# Autodesk Inventor assembly: KND-3600 Branch 6 01
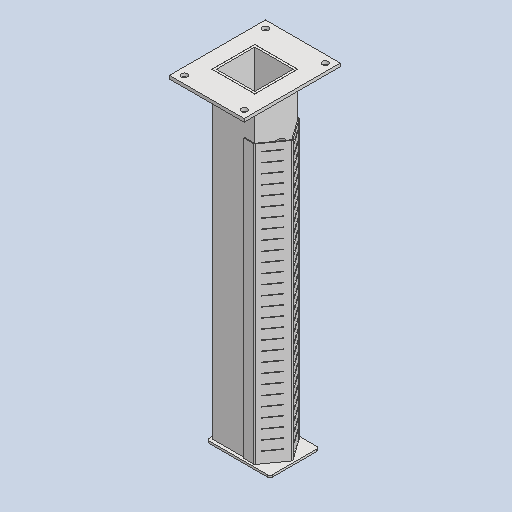
[picture p0: Inventor's stored thumbnail of the model, 512x512]
Saved by Autodesk Inventor 2026.2 (Build 302298000, 298)
## iProperties
Created: 2026-10-05
Part Number: KND-3600 Branch 6 01
Document SubType Name: Assembly
Designer: admin
Stock Number: Луч 6
Author: admin
## Documents named in this file (5)
- C:\Users\admin\Documents\Inventor\KND-DistribSystem\DRS_D1200\KND-3600 Branch 6 01.iam
- C:\Users\admin\Documents\Inventor\KND-DistribSystem\DRS_D1200\KND-1668 DrSysB way tube 6 01.ipt
- C:\Users\admin\Documents\Inventor\KND-DistribSystem\DRS_D1200\KND-1425 DrSysB Way FLANGE 01.ipt
- C:\Users\admin\Documents\Inventor\KND-DistribSystem\DRS_D1200\KND-5338 DrSysB roof 6 01.ipt
- C:\Users\admin\Documents\Inventor\KND-DistribSystem\DRS_D1200\KND-1666 FDS 1000 CUP 1 01.ipt
## Components (4 placed, 4 different names)
1. KND-1668 DrSysB way tube 6 01:1 — Flush:1, Mate:1, Mate:2, Flush:2, Mate:3, Mate:4, Mate:5, Flush:3, Flush:4
2. KND-1425 DrSysB Way FLANGE 01:1 — Flush:1, Mate:1, Mate:2
3. KND-5338 DrSysB roof 6 01:1 — Flush:2, Mate:3, Mate:4
4. KND-1666 FDS 1000 CUP 1 01:1 — Mate:5, Flush:3, Flush:4
## Relationships (9: Mate 5, Flush 4)
- Flush:1: KND-1668 DrSysB way tube 6 01:1 ↔ KND-1425 DrSysB Way FLANGE 01:1
- Mate:1 (0.1 mm): KND-1668 DrSysB way tube 6 01:1 ↔ KND-1425 DrSysB Way FLANGE 01:1
- Mate:2 (0.1 mm): KND-1668 DrSysB way tube 6 01:1 ↔ KND-1425 DrSysB Way FLANGE 01:1
- Flush:2: KND-1668 DrSysB way tube 6 01:1 ↔ KND-5338 DrSysB roof 6 01:1
- Mate:3 (0.1576 mm): KND-1668 DrSysB way tube 6 01:1 ↔ KND-5338 DrSysB roof 6 01:1
- Mate:4 (-9.5 mm): KND-1668 DrSysB way tube 6 01:1 ↔ KND-5338 DrSysB roof 6 01:1
- Mate:5: KND-1668 DrSysB way tube 6 01:1 ↔ KND-1666 FDS 1000 CUP 1 01:1
- Flush:3 (-3 mm): KND-1668 DrSysB way tube 6 01:1 ↔ KND-1666 FDS 1000 CUP 1 01:1
- Flush:4 (-2 mm): KND-1668 DrSysB way tube 6 01:1 ↔ KND-1666 FDS 1000 CUP 1 01:1
